# Autodesk Inventor assembly: Drone_Full
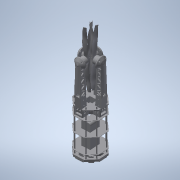
[picture p0: Inventor's stored thumbnail of the model, 180x180]
Saved by Autodesk Inventor 2020 (Build 240168000, 168)
## iProperties
Created: 2019-09-06
Part Number: Drone_Full
Document SubType Name: Assembly
Designer: isaac
Author: isaac
## Documents named in this file (11)
- C:\Users\User\Dropbox\IREC\Drone_Full.iam
- C:\Users\User\Dropbox\IREC\Arm Insert.ipt
- C:\Users\User\Dropbox\IREC\Arm.ipt
- C:\Users\User\Dropbox\IREC\Bottom.ipt
- C:\Users\User\Dropbox\IREC\Rod.ipt
- C:\Users\User\Dropbox\IREC\Top.ipt
- C:\Users\User\Dropbox\IREC\Layer.ipt
- C:\Users\User\Dropbox\IREC\Motor.ipt
- C:\Users\User\Dropbox\IREC\blade.ipt
- C:\Users\User\Dropbox\IREC\10000 mAh battery.ipt
- C:\Users\User\Dropbox\IREC\Camera.ipt
## Components (31 placed, 10 different names)
1. Arm Insert:1 — Mate:12, Flush:8, Mate:13, Mate:14, Mate:16
2. Arm:1 — Mate:12, Flush:8, Mate:14, Mate:41, Mate:42, Mate:43, Mate:60
3. Bottom:1 — Mate:2, Mate:11, Mate:15, Mate:55, Mate:56, Mate:57, Mate:58, Flush:13, Mate:59
4. Rod:1 — Mate:2, Mate:3, Flush:1, Mate:17, Mate:19, Mate:21
5. Top:1 — Mate:3, Mate:4, Mate:5, Mate:6, Mate:7, Mate:8, Mate:9, Mate:10, Mate:13, Mate:15, Mate:16, Mate:29, Mate:30, Mate:31, Mate:32, Mate:33, Mate:34, Flush:12, Mate:60, Mate:61
6. Rod:2 — Mate:4, Flush:1, Flush:3
7. Rod:3 — Mate:5, Flush:7, Mate:18, Mate:20, Mate:22
8. Rod:4 — Mate:6, Flush:6, Flush:7
9. Rod:5 — Mate:8, Flush:4, Flush:5, Mate:11
10. Rod:6 — Mate:9, Flush:2, Flush:4
11. Rod:7 — Mate:7, Flush:5, Flush:6
12. Rod:8 — Mate:10, Flush:2, Flush:3, Flush:12
13. Layer:1 — Mate:17, Mate:18
14. Layer:2 — Mate:19, Mate:20
15. Layer:3 — Mate:21, Mate:22
16. Arm Insert:2 — Mate:31, Mate:32
17. Arm:2 — Mate:35, Mate:36, Mate:37
18. Arm Insert:3 — Mate:30, Mate:33
19. Arm:3 — Mate:44, Mate:45, Mate:46
20. Arm Insert:4 — Mate:29, Mate:34
21. Arm:4 — Mate:38, Mate:39, Mate:40, Mate:61
22. Motor:1 — Mate:35, Mate:36, Mate:37, Mate:51, Mate:52
23. Motor:2 — Mate:38, Mate:39, Mate:40, Mate:49, Mate:50
24. Motor:3 — Mate:41, Mate:42, Mate:43, Mate:53, Mate:54
25. Motor:4 — Mate:44, Mate:45, Mate:46, Mate:47, Mate:48
26. blade:1 — Mate:47, Mate:48
27. blade:2 — Mate:49, Mate:50
28. blade:3 — Mate:51, Mate:52
29. blade:4 — Mate:53, Mate:54
30. 10000 mAh battery:1 — Mate:55, Mate:56, Mate:57
31. Camera:1 — Mate:58, Flush:13, Mate:59
## Relationships (73: Mate 60, Flush 13)
- Mate:2: Bottom:1 ↔ Rod:1
- Mate:3: Rod:1 ↔ Top:1
- Mate:4: Top:1 ↔ Rod:2
- Flush:1: Rod:1 ↔ Rod:2
- Mate:5: Top:1 ↔ Rod:3
- Mate:6: Top:1 ↔ Rod:4
- Mate:7: Top:1 ↔ Rod:7
- Mate:8: Top:1 ↔ Rod:5
- Mate:9: Top:1 ↔ Rod:6
- Mate:10: Top:1 ↔ Rod:8
- Flush:2: Rod:6 ↔ Rod:8
- Flush:3: Rod:2 ↔ Rod:8
- Flush:4: Rod:5 ↔ Rod:6
- Flush:5: Rod:5 ↔ Rod:7
- Flush:6: Rod:4 ↔ Rod:7
- Flush:7: Rod:3 ↔ Rod:4
- Mate:11: Bottom:1 ↔ Rod:5
- Mate:12: Arm Insert:1 ↔ Arm:1
- Flush:8: Arm Insert:1 ↔ Arm:1
- Mate:13: Arm Insert:1 ↔ Top:1
- Mate:14: Arm Insert:1 ↔ Arm:1
- Mate:15 (228.6 mm): Bottom:1 ↔ Top:1
- Mate:16 (0.3969 mm): Arm Insert:1 ↔ Top:1
- Mate:17: Rod:1 ↔ Layer:1
- Mate:18: Rod:3 ↔ Layer:1
- Mate:19: Rod:1 ↔ Layer:2
- Mate:20: Rod:3 ↔ Layer:2
- Mate:21: Rod:1 ↔ Layer:3
- Mate:22: Rod:3 ↔ Layer:3
- [Mate]: Arm Insert:2 ↔ Arm:2
- [Flush]: Arm Insert:2 ↔ Arm:2
- [Mate]: Arm Insert:2 ↔ Arm:2
- [Mate]: Arm Insert:3 ↔ Arm:3
- [Flush]: Arm Insert:3 ↔ Arm:3
- [Mate]: Arm Insert:3 ↔ Arm:3
- [Mate]: Arm Insert:4 ↔ Arm:4
- [Flush]: Arm Insert:4 ↔ Arm:4
- [Mate]: Arm Insert:4 ↔ Arm:4
- Mate:29: Top:1 ↔ Arm Insert:4
- Mate:30: Top:1 ↔ Arm Insert:3
- Mate:31 (0.3969 mm): Top:1 ↔ Arm Insert:2
- Mate:32: Top:1 ↔ Arm Insert:2
- Mate:33: Top:1 ↔ Arm Insert:3
- Mate:34: Top:1 ↔ Arm Insert:4
- Flush:12 (-12.7 mm): Top:1 ↔ Rod:8
- Mate:35: Arm:2 ↔ Motor:1
- Mate:36: Arm:2 ↔ Motor:1
- Mate:37: Arm:2 ↔ Motor:1
- Mate:38: Arm:4 ↔ Motor:2
- Mate:39: Arm:4 ↔ Motor:2
- Mate:40: Arm:4 ↔ Motor:2
- Mate:41: Arm:1 ↔ Motor:3
- Mate:42: Arm:1 ↔ Motor:3
- Mate:43: Arm:1 ↔ Motor:3
- Mate:44: Arm:3 ↔ Motor:4
- Mate:45: Arm:3 ↔ Motor:4
- Mate:46: Arm:3 ↔ Motor:4
- Mate:47: Motor:4 ↔ blade:1
- Mate:48: Motor:4 ↔ blade:1
- Mate:49: Motor:2 ↔ blade:2
- Mate:50: Motor:2 ↔ blade:2
- Mate:51: Motor:1 ↔ blade:3
- Mate:52: Motor:1 ↔ blade:3
- Mate:53: Motor:3 ↔ blade:4
- Mate:54: Motor:3 ↔ blade:4
- Mate:55: Bottom:1 ↔ 10000 mAh battery:1
- Mate:56: Bottom:1 ↔ 10000 mAh battery:1
- Mate:57: Bottom:1 ↔ 10000 mAh battery:1
- Mate:58: Bottom:1 ↔ Camera:1
- Flush:13: Bottom:1 ↔ Camera:1
- Mate:59: Bottom:1 ↔ Camera:1
- Mate:60: Arm:1 ↔ Top:1
- Mate:61: Top:1 ↔ Arm:4
## Named parameters: d32_d20 = 0 mm, d33_d21 = 0 mm, d34_d23 = 0 mm, d35_d20 = 0 mm, d36_d21 = 0 mm, d37_d23 = 0 mm, d38_d20 = 0 mm, d39_d21 = 0 mm, d40_d23 = 0 mm
